# Autodesk Inventor assembly: Ensamblaje1
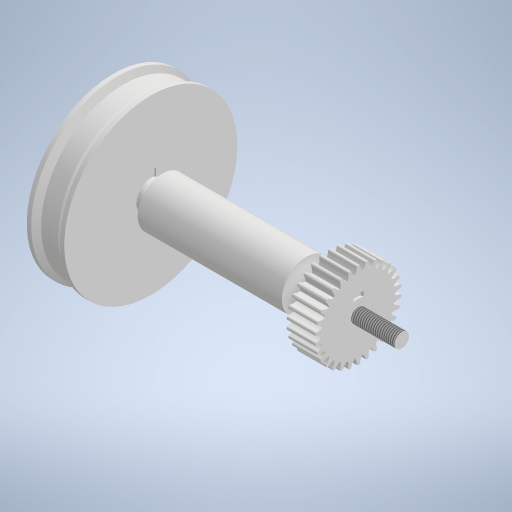
[picture p0: Inventor's stored thumbnail of the model, 512x512]
Saved by Autodesk Inventor 2024 (Build 280153000, 153)
## iProperties
Created: 2024-03-17
Part Number: Ensamblaje1
Document SubType Name: Assembly
Designer: joelm
Author: joelm
## Documents named in this file (6)
- C:\Users\joelm\Documents\Inventor 2024\Bin\Ensamblaje1.iam
- C:\Users\joelm\Downloads\ENGRANE.ipt
- C:\Users\joelm\Downloads\POLEA.ipt
- C:\Users\joelm\Downloads\EJE_CUÑEROS.ipt
- C:\Users\joelm\Downloads\CUÑA.ipt
- C:\Users\joelm\Downloads\rosca ensamble.ipt
## Components (6 placed, 5 different names)
1. ENGRANE:1 — Rígido:3, Nivelación:2, Nivelación:3, Nivelación:4, Nivelación:5
2. POLEA:1 — Cilíndrica:1, Nivelación:1
3. EJE_CUÑEROS:1 — Cilíndrica:1, Rígido:1, Rígido:2, Rígido:3, Nivelación:3, De rotación:1
4. CUÑA:1 — Rígido:1, Nivelación:1
5. CUÑA:2 — Rígido:2, Nivelación:2, Nivelación:4, Nivelación:5
6. rosca ensamble:1 — De rotación:1
## Relationships (10: Flush 5, WeldJoint 3, CylindricalJoint 1, RevoluteJoint 1)
- Cilíndrica:1 [CylindricalJoint]: POLEA:1 ↔ EJE_CUÑEROS:1
- Rígido:1 [WeldJoint]: EJE_CUÑEROS:1 ↔ CUÑA:1
- Nivelación:1 [Flush]: POLEA:1 ↔ CUÑA:1
- Rígido:2 [WeldJoint]: EJE_CUÑEROS:1 ↔ CUÑA:2
- Rígido:3 [WeldJoint]: ENGRANE:1 ↔ EJE_CUÑEROS:1
- Nivelación:2 [Flush]: ENGRANE:1 ↔ CUÑA:2
- Nivelación:3 [Flush]: ENGRANE:1 ↔ EJE_CUÑEROS:1
- Nivelación:4 [Flush]: ENGRANE:1 ↔ CUÑA:2
- Nivelación:5 [Flush]: ENGRANE:1 ↔ CUÑA:2
- De rotación:1 [RevoluteJoint]: EJE_CUÑEROS:1 ↔ rosca ensamble:1
